# Autodesk Inventor assembly: base_ass_4
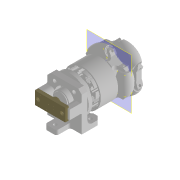
[picture p0: Inventor's stored thumbnail of the model, 180x180]
Saved by Autodesk Inventor 2020 (Build 240168000, 168)
## iProperties
Created: 2022-01-21
Part Number: base_ass_4
Document SubType Name: Assembly
Designer: Shuang Peng
Author: Shuang Peng
## Documents named in this file (6)
- D:\projects-3\soft module robot\hardware\diff module 3\base_ass_4.iam
- D:\projects-3\soft module robot\hardware\diff module 3\motor_1613_3.iam
- D:\projects-3\soft module robot\hardware\diff module 3\ma_holder_1.ipt
- D:\projects-3\soft module robot\hardware\diff module 3\encoder_ma_6_2.5.ipt
- D:\projects-3\soft module robot\hardware\diff module 3\Board.ipt
- D:\projects-3\soft module robot\hardware\diff module 3\motor_hl_1.ipt
## Components (5 placed, 5 different names)
1. motor_1613_3:1 [sub-assembly] — Angle:1, Insert:5, Insert:6, Insert:7
2. ma_holder_1:1 — Insert:5
3. encoder_ma_6_2.5:1 — Insert:4
4. Board:1 — Insert:4, Angle:1
5. motor_hl_1:1 — Insert:6, Insert:7
## Relationships (6: Insert 5, Angle 1)
- [Insert]: ma_holder_1:1 ↔ encoder_ma_6_2.5:1
- Insert:4 (1.5 mm): encoder_ma_6_2.5:1 ↔ Board:1
- Angle:1 (0 deg): motor_1613_3:1 ↔ Board:1
- Insert:5: motor_1613_3:1 ↔ ma_holder_1:1
- Insert:6: motor_1613_3:1 ↔ motor_hl_1:1
- Insert:7: motor_1613_3:1 ↔ motor_hl_1:1
## Named parameters: d18_d17 = 0 mm
